# Autodesk Inventor assembly: componentBallRamp
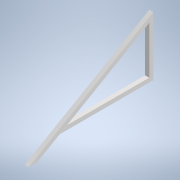
[picture p0: Inventor's stored thumbnail of the model, 180x180]
Saved by Autodesk Inventor 2020.2 (Build 242310000, 310)
## iProperties
Created: 2020-01-19
Part Number: componentBallRamp
Document SubType Name: Assembly
Designer: robst
Author: robst
## Documents named in this file (4)
- C:\git\CAD-Development\robSteele\2020BallTriggerMechanism\componentBallRamp.iam
- C:\git\CAD-Development\robSteele\2020BallTriggerMechanism\baseAluminumExtrusion.ipt
- C:\git\CAD-Development\robSteele\2020BallTriggerMechanism\sideAluminumExtrusion.ipt
- C:\git\CAD-Development\robSteele\2020BallTriggerMechanism\hypotAluminumExtrusion.ipt
## Components (3 placed, 3 different names)
1. baseAluminumExtrusion:1 — Mate:1, Flush:1, Flush:2
2. sideAluminumExtrusion:1 — Mate:1, Flush:1, Flush:2, Mate:2, Flush:3, Mate:3
3. hypotAluminumExtrusion:1 — Mate:2, Flush:3, Mate:3
## Relationships (6: Mate 3, Flush 3)
- Mate:1: baseAluminumExtrusion:1 ↔ sideAluminumExtrusion:1
- Flush:1: baseAluminumExtrusion:1 ↔ sideAluminumExtrusion:1
- Flush:2: baseAluminumExtrusion:1 ↔ sideAluminumExtrusion:1
- Mate:2: sideAluminumExtrusion:1 ↔ hypotAluminumExtrusion:1
- Flush:3: sideAluminumExtrusion:1 ↔ hypotAluminumExtrusion:1
- Mate:3: sideAluminumExtrusion:1 ↔ hypotAluminumExtrusion:1
